# Autodesk Inventor assembly: MMAE 232 CAD Assignment 2 Servo Assembly-Nicholas Skiba
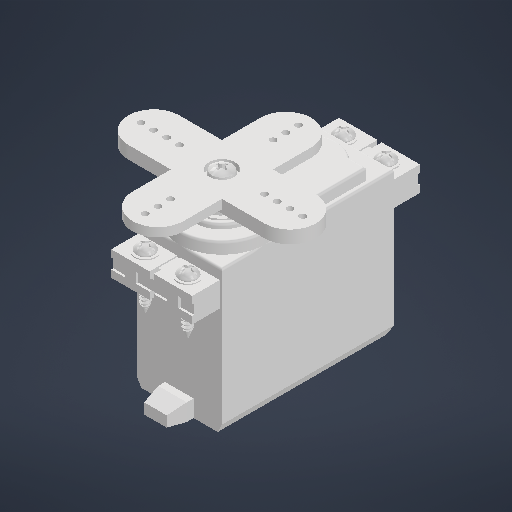
[picture p0: Inventor's stored thumbnail of the model, 512x512]
Saved by Autodesk Inventor 2026.1 (Build 301233000, 233)
## iProperties
Created: 2025-08-29
Part Number: MMAE 232 CAD Assignment 2 Servo Assembly-Nicholas Skiba
Document SubType Name: Assembly
Designer: Nick
Author: Nick
## Documents named in this file (7)
- C:\Users\Nick\Downloads\CAD\Inventor\MMAE 232 Homeworks\CAD 2\MMAE 232 CAD Assignment 2 Servo Assembly-Nicholas Skiba.iam
- C:\Users\Nick\Downloads\CAD\Inventor\MMAE 232 Homeworks\CAD 2\MMAE 232 CAD Assignment 2 Servo-Nicholas Skiba.ipt
- C:\Users\Nick\Downloads\CAD\Inventor\MMAE 232 Homeworks\CAD 2\MMAE 232 CAD Assignment 2 Rubber Grommet-Nicholas Skiba.ipt
- C:\Users\Nick\Downloads\CAD\Inventor\MMAE 232 Homeworks\CAD 2\MMAE 232 CAD Assignment 2 Brass Sleeve-Nicholas Skiba.ipt
- C:\Users\Nick\Downloads\CAD\Inventor\MMAE 232 Homeworks\CAD 2\MMAE 232 CAD Assignment 2 Servo Horn 3-Nicholas Skiba.ipt
- C:\Users\Nick\Downloads\CAD\Inventor\MMAE 232 Homeworks\CAD 2\90184A064_Phillips Rounded Head Screws for Sheet Metal.ipt
- C:\Users\Nick\Downloads\CAD\Inventor\MMAE 232 Homeworks\CAD 2\95836A255_Black-Oxide 18-8 Stainless Steel Pan Hea.ipt
## Components (15 placed, 6 different names)
1. MMAE 232 CAD Assignment 2 Servo-Nicholas Skiba:1 — Mate:1, Mate:2, Mate:3, Mate:4, Mate:5, Mate:6, Mate:7, Mate:8, Mate:9, Mate:10, Mate:11, Mate:12, Mate:21, Mate:22
2. MMAE 232 CAD Assignment 2 Rubber Grommet-Nicholas Skiba:1 — Mate:10, Mate:11, Mate:12, Mate:19, Mate:20
3. MMAE 232 CAD Assignment 2 Rubber Grommet-Nicholas Skiba:2 — Mate:4, Mate:5, Mate:6, Mate:15, Mate:16
4. MMAE 232 CAD Assignment 2 Rubber Grommet-Nicholas Skiba:3 — Mate:1, Mate:2, Mate:3, Mate:13, Mate:14
5. MMAE 232 CAD Assignment 2 Rubber Grommet-Nicholas Skiba:4 — Mate:7, Mate:8, Mate:9, Mate:17, Mate:18
6. MMAE 232 CAD Assignment 2 Brass Sleeve-Nicholas Skiba:1 — Mate:15, Mate:16, Mate:23, Mate:24
7. MMAE 232 CAD Assignment 2 Brass Sleeve-Nicholas Skiba:2 — Mate:13, Mate:14, Mate:25, Mate:26
8. MMAE 232 CAD Assignment 2 Brass Sleeve-Nicholas Skiba:3 — Mate:19, Mate:20, Mate:28, Mate:29
9. MMAE 232 CAD Assignment 2 Brass Sleeve-Nicholas Skiba:4 — Mate:17, Mate:18, Mate:27, Mate:30
10. MMAE 232 CAD Assignment 2 Servo Horn 3-Nicholas Skiba:1 — Mate:21, Mate:22, Mate:31, Mate:32
11. 90184A064_Phillips Rounded Head Screws for Sheet Metal:1 — Mate:28, Mate:29
12. 90184A064_Phillips Rounded Head Screws for Sheet Metal:2 — Mate:23, Mate:24
13. 90184A064_Phillips Rounded Head Screws for Sheet Metal:3 — Mate:27, Mate:30
14. 90184A064_Phillips Rounded Head Screws for Sheet Metal:4 — Mate:25, Mate:26
15. 95836A255_Black-Oxide 18-8 Stainless Steel Pan Hea:1 — Mate:31, Mate:32
## Relationships (32: Mate 32)
- Mate:1: MMAE 232 CAD Assignment 2 Servo-Nicholas Skiba:1 ↔ MMAE 232 CAD Assignment 2 Rubber Grommet-Nicholas Skiba:3
- Mate:2: MMAE 232 CAD Assignment 2 Servo-Nicholas Skiba:1 ↔ MMAE 232 CAD Assignment 2 Rubber Grommet-Nicholas Skiba:3
- Mate:3: MMAE 232 CAD Assignment 2 Servo-Nicholas Skiba:1 ↔ MMAE 232 CAD Assignment 2 Rubber Grommet-Nicholas Skiba:3
- Mate:4: MMAE 232 CAD Assignment 2 Servo-Nicholas Skiba:1 ↔ MMAE 232 CAD Assignment 2 Rubber Grommet-Nicholas Skiba:2
- Mate:5: MMAE 232 CAD Assignment 2 Servo-Nicholas Skiba:1 ↔ MMAE 232 CAD Assignment 2 Rubber Grommet-Nicholas Skiba:2
- Mate:6: MMAE 232 CAD Assignment 2 Servo-Nicholas Skiba:1 ↔ MMAE 232 CAD Assignment 2 Rubber Grommet-Nicholas Skiba:2
- Mate:7: MMAE 232 CAD Assignment 2 Servo-Nicholas Skiba:1 ↔ MMAE 232 CAD Assignment 2 Rubber Grommet-Nicholas Skiba:4
- Mate:8: MMAE 232 CAD Assignment 2 Servo-Nicholas Skiba:1 ↔ MMAE 232 CAD Assignment 2 Rubber Grommet-Nicholas Skiba:4
- Mate:9: MMAE 232 CAD Assignment 2 Servo-Nicholas Skiba:1 ↔ MMAE 232 CAD Assignment 2 Rubber Grommet-Nicholas Skiba:4
- Mate:10: MMAE 232 CAD Assignment 2 Servo-Nicholas Skiba:1 ↔ MMAE 232 CAD Assignment 2 Rubber Grommet-Nicholas Skiba:1
- Mate:11: MMAE 232 CAD Assignment 2 Servo-Nicholas Skiba:1 ↔ MMAE 232 CAD Assignment 2 Rubber Grommet-Nicholas Skiba:1
- Mate:12: MMAE 232 CAD Assignment 2 Servo-Nicholas Skiba:1 ↔ MMAE 232 CAD Assignment 2 Rubber Grommet-Nicholas Skiba:1
- Mate:13: MMAE 232 CAD Assignment 2 Rubber Grommet-Nicholas Skiba:3 ↔ MMAE 232 CAD Assignment 2 Brass Sleeve-Nicholas Skiba:2
- Mate:14: MMAE 232 CAD Assignment 2 Rubber Grommet-Nicholas Skiba:3 ↔ MMAE 232 CAD Assignment 2 Brass Sleeve-Nicholas Skiba:2
- Mate:15: MMAE 232 CAD Assignment 2 Rubber Grommet-Nicholas Skiba:2 ↔ MMAE 232 CAD Assignment 2 Brass Sleeve-Nicholas Skiba:1
- Mate:16: MMAE 232 CAD Assignment 2 Rubber Grommet-Nicholas Skiba:2 ↔ MMAE 232 CAD Assignment 2 Brass Sleeve-Nicholas Skiba:1
- Mate:17: MMAE 232 CAD Assignment 2 Rubber Grommet-Nicholas Skiba:4 ↔ MMAE 232 CAD Assignment 2 Brass Sleeve-Nicholas Skiba:4
- Mate:18: MMAE 232 CAD Assignment 2 Rubber Grommet-Nicholas Skiba:4 ↔ MMAE 232 CAD Assignment 2 Brass Sleeve-Nicholas Skiba:4
- Mate:19: MMAE 232 CAD Assignment 2 Rubber Grommet-Nicholas Skiba:1 ↔ MMAE 232 CAD Assignment 2 Brass Sleeve-Nicholas Skiba:3
- Mate:20: MMAE 232 CAD Assignment 2 Rubber Grommet-Nicholas Skiba:1 ↔ MMAE 232 CAD Assignment 2 Brass Sleeve-Nicholas Skiba:3
- Mate:21: MMAE 232 CAD Assignment 2 Servo-Nicholas Skiba:1 ↔ MMAE 232 CAD Assignment 2 Servo Horn 3-Nicholas Skiba:1
- Mate:22: MMAE 232 CAD Assignment 2 Servo-Nicholas Skiba:1 ↔ MMAE 232 CAD Assignment 2 Servo Horn 3-Nicholas Skiba:1
- Mate:23: MMAE 232 CAD Assignment 2 Brass Sleeve-Nicholas Skiba:1 ↔ 90184A064_Phillips Rounded Head Screws for Sheet Metal:2
- Mate:24: MMAE 232 CAD Assignment 2 Brass Sleeve-Nicholas Skiba:1 ↔ 90184A064_Phillips Rounded Head Screws for Sheet Metal:2
- Mate:25: MMAE 232 CAD Assignment 2 Brass Sleeve-Nicholas Skiba:2 ↔ 90184A064_Phillips Rounded Head Screws for Sheet Metal:4
- Mate:26: MMAE 232 CAD Assignment 2 Brass Sleeve-Nicholas Skiba:2 ↔ 90184A064_Phillips Rounded Head Screws for Sheet Metal:4
- Mate:27: MMAE 232 CAD Assignment 2 Brass Sleeve-Nicholas Skiba:4 ↔ 90184A064_Phillips Rounded Head Screws for Sheet Metal:3
- Mate:28: MMAE 232 CAD Assignment 2 Brass Sleeve-Nicholas Skiba:3 ↔ 90184A064_Phillips Rounded Head Screws for Sheet Metal:1
- Mate:29: MMAE 232 CAD Assignment 2 Brass Sleeve-Nicholas Skiba:3 ↔ 90184A064_Phillips Rounded Head Screws for Sheet Metal:1
- Mate:30: MMAE 232 CAD Assignment 2 Brass Sleeve-Nicholas Skiba:4 ↔ 90184A064_Phillips Rounded Head Screws for Sheet Metal:3
- Mate:31: MMAE 232 CAD Assignment 2 Servo Horn 3-Nicholas Skiba:1 ↔ 95836A255_Black-Oxide 18-8 Stainless Steel Pan Hea:1
- Mate:32: MMAE 232 CAD Assignment 2 Servo Horn 3-Nicholas Skiba:1 ↔ 95836A255_Black-Oxide 18-8 Stainless Steel Pan Hea:1
